# Autodesk Inventor assembly: SampleSetup
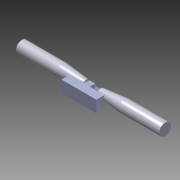
[picture p0: Inventor's stored thumbnail of the model, 180x180]
Saved by Autodesk Inventor 2015 (Build 190159000, 159)
## iProperties
Created: 2015-02-01
Part Number: SampleSetup
Document SubType Name: Assembly
Designer: Paul
Author: Paul
## Documents named in this file (4)
- C:\Users\Paul\Google Drive\All #ResBaz Shared\Paul2AlizaCAD\05_Assemby\Files\02_SampleHolder\SHolder_Answer.iam
- C:\Users\Paul\Google Drive\All #ResBaz Shared\Paul2AlizaCAD\05_Assemby\Files\02_SampleHolder\Sample_Holder.ipt
- C:\Users\Paul\Google Drive\All #ResBaz Shared\Paul2AlizaCAD\05_Assemby\Files\02_SampleHolder\Sample.ipt
- C:\Users\Paul\Google Drive\All #ResBaz Shared\Paul2AlizaCAD\05_Assemby\Files\02_SampleHolder\Support.ipt
## Components (4 placed, 3 different names)
1. Sample_Holder:1 — Mate:1, Flush:3
2. Sample:1 — Mate:1, Flush:3, Mate:2, Mate:3, Mate:4, Mate:5
3. Support:1 — Mate:2, Mate:4
4. Support:2 — Mate:3, Mate:5
## Relationships (6: Mate 5, Flush 1)
- Mate:1: Sample_Holder:1 ↔ Sample:1
- Flush:3 (-7.5 mm): Sample_Holder:1 ↔ Sample:1
- Mate:2: Sample:1 ↔ Support:1
- Mate:3: Sample:1 ↔ Support:2
- Mate:4: Sample:1 ↔ Support:1
- Mate:5: Sample:1 ↔ Support:2
